# Autodesk Inventor assembly: каркас странный
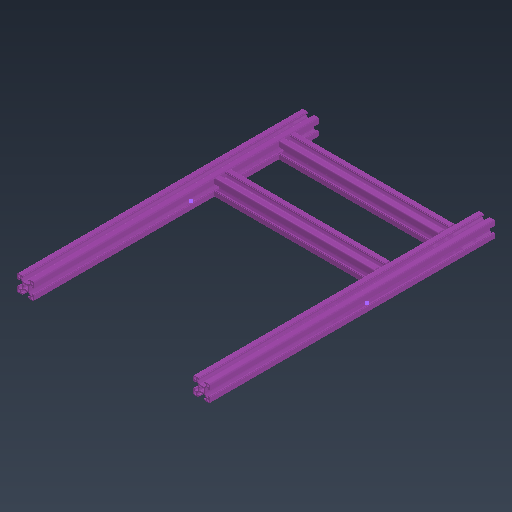
[picture p0: Inventor's stored thumbnail of the model, 512x512]
Saved by Autodesk Inventor 2025 (Build 290162000, 162)
## iProperties
Created: 2025-01-29
Part Number: каркас странный
Document SubType Name: Assembly
Designer: GameHD
Author: GameHD
## Documents named in this file (3)
- C:\Users\GameHD\Desktop\phantom 16950\каркас странный.iam
- C:\Users\GameHD\Desktop\phantom 16950\профиль каркас.ipt
- C:\Users\GameHD\Desktop\phantom 16950\профиль каркас паралельно.ipt
## Components (4 placed, 2 different names)
1. профиль каркас:1
2. профиль каркас паралельно:1
3. профиль каркас паралельно:2
4. профиль каркас:2
## Relationships (6: Mate 3, Flush 3)
- [Mate]: профиль каркас:1 ↔ профиль каркас паралельно:1
- [Flush]: профиль каркас:1 ↔ профиль каркас паралельно:1
- [Mate]: профиль каркас:1 ↔ профиль каркас паралельно:2
- [Flush]: профиль каркас:1 ↔ профиль каркас паралельно:2
- [Mate]: профиль каркас паралельно:1 ↔ профиль каркас:2
- [Flush]: профиль каркас:1 ↔ профиль каркас:2
